# Autodesk Inventor assembly: nanotwister_reaper
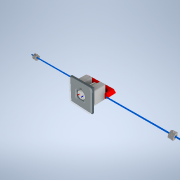
[picture p0: Inventor's stored thumbnail of the model, 180x180]
Saved by Autodesk Inventor 2021 (Build 250183000, 183)
## iProperties
Created: 2022-02-27
Part Number: nanotwister_reaper
Document SubType Name: Assembly
Designer: ermoz
Author: ermoz
## Documents named in this file (8)
- D:\Moje Wyczyny\My_Poor_Projects\nanosumo-nanotwister\mechanics\nanotwister_reaper.iam
- D:\Moje Wyczyny\My_Poor_Projects\nanosumo-nanotwister\mechanics\motor_noname.ipt
- D:\Moje Wyczyny\My_Poor_Projects\nanosumo-nanotwister\mechanics\pb_hole.ipt
- D:\Moje Wyczyny\My_Poor_Projects\nanosumo-nanotwister\mechanics\hot_glue_mashroom.ipt
- D:\Moje Wyczyny\My_Poor_Projects\nanosumo-nanotwister\mechanics\battery_1S_100mAh_no_prot.ipt
- D:\Moje Wyczyny\My_Poor_Projects\nanosumo-nanotwister\mechanics\rotor_core.ipt
- D:\Moje Wyczyny\My_Poor_Projects\nanosumo-nanotwister\mechanics\3M_Nut.ipt
- D:\Moje Wyczyny\My_Poor_Projects\nanosumo-nanotwister\mechanics\wire.ipt
## Components (12 placed, 7 different names)
1. motor_noname:1 — Mate:1, Mate:5, Tangent:1, Tangent:2, Mate:8, Flush:4
2. pb_hole:1 — Mate:1, Mate:4, Flush:2, Flush:3, Mate:6, Mate:7, Angle:1, Angle:2, Angle:3
3. hot_glue_mashroom:1 — Mate:4, Flush:2, Flush:3, Mate:5
4. battery_1S_100mAh_no_prot:1 — Mate:6, Tangent:1, Angle:1
5. battery_1S_100mAh_no_prot:2 — Mate:7, Tangent:2, Angle:2
6. rotor_core:1 — Mate:8, Flush:4, Angle:3, Tangent:5, Mate:18, Angle:4, Tangent:6, Tangent:7
7. 3M_Nut:1 — Mate:12, Mate:16
8. 3M_Nut:2 — Mate:11, Flush:6, Mate:16
9. 3M_Nut:3 — Mate:13, Mate:15
10. 3M_Nut:4 — Mate:14, Flush:5, Mate:15
11. wire:1 — Mate:11, Mate:12, Flush:6, Mate:17, Tangent:5, Tangent:6, Tangent:8
12. wire:2 — Mate:13, Mate:14, Flush:5, Mate:17, Tangent:7
## Relationships (29: Mate 14, Tangent 6, Flush 5, Angle 4)
- Mate:1: motor_noname:1 ↔ pb_hole:1
- Mate:4: pb_hole:1 ↔ hot_glue_mashroom:1
- Flush:2 (0.25 mm): pb_hole:1 ↔ hot_glue_mashroom:1
- Flush:3 (0.25 mm): pb_hole:1 ↔ hot_glue_mashroom:1
- Mate:5: motor_noname:1 ↔ hot_glue_mashroom:1
- Mate:6: pb_hole:1 ↔ battery_1S_100mAh_no_prot:1
- Mate:7: pb_hole:1 ↔ battery_1S_100mAh_no_prot:2
- Tangent:1: motor_noname:1 ↔ battery_1S_100mAh_no_prot:1
- Tangent:2: motor_noname:1 ↔ battery_1S_100mAh_no_prot:2
- Angle:1 (0 deg): pb_hole:1 ↔ battery_1S_100mAh_no_prot:1
- Angle:2 (0 deg): pb_hole:1 ↔ battery_1S_100mAh_no_prot:2
- Mate:8: motor_noname:1 ↔ rotor_core:1
- Flush:4: motor_noname:1 ↔ rotor_core:1
- Mate:11: 3M_Nut:2 ↔ wire:1
- Mate:12: 3M_Nut:1 ↔ wire:1
- Mate:13: 3M_Nut:3 ↔ wire:2
- Mate:14: 3M_Nut:4 ↔ wire:2
- Flush:5 (-5 mm): 3M_Nut:4 ↔ wire:2
- Mate:15: 3M_Nut:3 ↔ 3M_Nut:4
- Flush:6 (5 mm): 3M_Nut:2 ↔ wire:1
- Mate:16: 3M_Nut:1 ↔ 3M_Nut:2
- Angle:3 (360 deg): pb_hole:1 ↔ rotor_core:1
- Mate:17: wire:1 ↔ wire:2
- Tangent:5: rotor_core:1 ↔ wire:1
- Mate:18: rotor_core:1
- Angle:4 (0 deg): rotor_core:1
- Tangent:6: rotor_core:1 ↔ wire:1
- Tangent:7: rotor_core:1 ↔ wire:2
- Tangent:8 (-0.6 mm): wire:1
